# Autodesk Inventor assembly: Ensamblaje_tesis
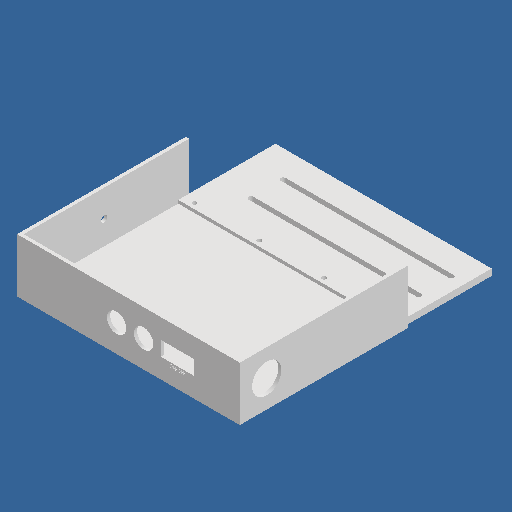
[picture p0: Inventor's stored thumbnail of the model, 512x512]
Saved by Autodesk Inventor 2025 (Build 290162000, 162)
## iProperties
Created: 2026-01-02
Part Number: Ensamblaje_tesis
Document SubType Name: Assembly
Designer: HP
Author: HP
## Documents named in this file (3)
- C:\Users\HP\Desktop\TESIS 2\TFC2_20212123_MHinojosa\TFC2-20212123-HW\CAD\Ensamblaje_tesis.iam
- C:\Users\HP\Desktop\TESIS 2\TFC2_20212123_MHinojosa\TFC2-20212123-HW\CAD\MesaDePruebas.ipt
- C:\Users\HP\Desktop\TESIS 2\TFC2_20212123_MHinojosa\TFC2-20212123-HW\CAD\Chasis.ipt
## Components (2 placed, 2 different names)
1. MesaDePruebas:1 — Nivelación:1, Coincidencia:1, Coincidencia:2
2. Chasis:1 — Nivelación:1, Coincidencia:1, Coincidencia:2
## Relationships (3: Mate 2, Flush 1)
- Nivelación:1 [Flush]: MesaDePruebas:1 ↔ Chasis:1
- Coincidencia:1 [Mate]: MesaDePruebas:1 ↔ Chasis:1
- Coincidencia:2 [Mate]: MesaDePruebas:1 ↔ Chasis:1
